# Autodesk Inventor assembly: Assembly2
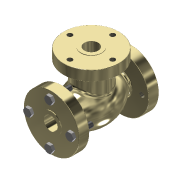
[picture p0: Inventor's stored thumbnail of the model, 180x180]
Saved by Autodesk Inventor 2019 (Build 230136000, 136)
## iProperties
Created: 2023-07-05
Part Number: Assembly2
Document SubType Name: Assembly
Designer: Fransic
Author: Fransic
## Documents named in this file (4)
- C:\Users\Fransic\Documents\Inventor\Shock Absorber\Assembly2.iam
- C:\Users\Fransic\Documents\PERSONAL DOCUMENT\GLOBE VALVE\BODY.ipt
- C:\Users\Fransic\Documents\Inventor\Content Center Files\R2019\en-US\DIN EN ISO 4014\DIN EN ISO 4014 - M18 x 70.ipt
- C:\Users\Fransic\Documents\Inventor\Content Center Files\R2019\en-US\ANSI B18.22 M\ANSI B18.22M - 20 N.ipt
## Components (10 placed, 3 different names)
1. BODY:1 — Insert:1, Insert:2, Insert:3, Insert:4, Mate:2, Insert:5, Insert:6, Insert:7, Insert:8
2. DIN EN ISO 4014 M18 x 70:1 — Insert:1
3. DIN EN ISO 4014 M18 x 70:2 — Insert:2, Mate:1
4. DIN EN ISO 4014 M18 x 70:3 — Insert:3
5. DIN EN ISO 4014 M18 x 70:4 — Insert:4
6. Plain Washer (Metric) 20 N:1 — Mate:1, Mate:2
7. Plain Washer (Metric) 20 N:2 — Insert:5
8. Plain Washer (Metric) 20 N:3 — Insert:6
9. Plain Washer (Metric) 20 N:4 — Insert:7
10. Plain Washer (Metric) 20 N:5 — Insert:8
## Relationships (10: Insert 8, Mate 2)
- Insert:1: BODY:1 ↔ DIN EN ISO 4014 M18 x 70:1
- Insert:2: BODY:1 ↔ DIN EN ISO 4014 M18 x 70:2
- Insert:3: BODY:1 ↔ DIN EN ISO 4014 M18 x 70:3
- Insert:4: BODY:1 ↔ DIN EN ISO 4014 M18 x 70:4
- Mate:1: DIN EN ISO 4014 M18 x 70:2 ↔ Plain Washer (Metric) 20 N:1
- Mate:2: BODY:1 ↔ Plain Washer (Metric) 20 N:1
- Insert:5: BODY:1 ↔ Plain Washer (Metric) 20 N:2
- Insert:6: BODY:1 ↔ Plain Washer (Metric) 20 N:3
- Insert:7: BODY:1 ↔ Plain Washer (Metric) 20 N:4
- Insert:8: BODY:1 ↔ Plain Washer (Metric) 20 N:5
